# Autodesk Inventor assembly: CF70_nipple_Membrane
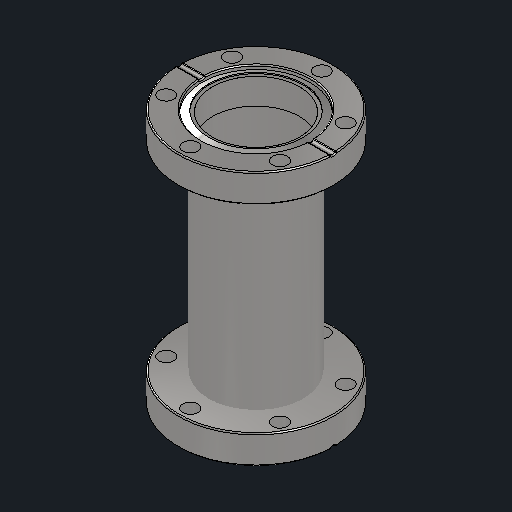
[picture p0: Inventor's stored thumbnail of the model, 512x512]
Saved by Autodesk Inventor 2026 (Build 300175050, 175E)
## iProperties
Created: 2022-11-16
Part Number: CF70_nipple_Membrane
Document SubType Name: Assembly
Designer: kuzmin
Mass: 550.715 g
Surface Area: 368.58 cm^2
Volume: 71.06 cm^3
Density: 7.75 g/cm^3
Author: kuzmin
## Documents named in this file (3)
- C:\Users\queez\Dropbox\Drawings\PIHTI\ContentCenter\CF-parts\CF70-nipple\CF70-nipple.iam
- C:\Users\queez\Dropbox\Drawings\PIHTI\ContentCenter\CF-parts\CF70-nipple\cf70_hole_nipple.ipt
- C:\Users\queez\Dropbox\Drawings\PIHTI\ContentCenter\CF-parts\CF70-nipple\CF70_nipple_Membrane.ipt
## Components (3 placed, 2 different names)
1. cf70_hole_nipple:1 — Mate:1, Flush:1, Mate:3
2. cf70_hole_nipple:2 — Mate:2, Flush:2, Mate:3
3. CF70_nipple_Membrane:1 — Mate:1, Mate:2, Flush:1, Flush:2
## Relationships (5: Mate 3, Flush 2)
- Mate:1: cf70_hole_nipple:1 ↔ CF70_nipple_Membrane:1
- Mate:2: cf70_hole_nipple:2 ↔ CF70_nipple_Membrane:1
- Flush:1: cf70_hole_nipple:1 ↔ CF70_nipple_Membrane:1
- Flush:2: cf70_hole_nipple:2 ↔ CF70_nipple_Membrane:1
- Mate:3 (-114 mm): cf70_hole_nipple:1 ↔ cf70_hole_nipple:2
